# Autodesk Inventor assembly: Assembly_ball_test
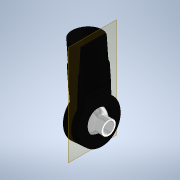
[picture p0: Inventor's stored thumbnail of the model, 180x180]
Saved by Autodesk Inventor 2020 (Build 240168000, 168)
## iProperties
Created: 2019-11-09
Part Number: Assembly_ball_test
Document SubType Name: Assembly
Designer: maste
Author: maste
## Documents named in this file (3)
- C:\Users\maste\Documents\GitHub\autobot\robot_model\Assembly_ball_test.iam
- C:\Users\maste\Documents\GitHub\autobot\robot_model\RCT-H017_Bola_de_libertad_menor.ipt
- C:\Users\maste\Documents\GitHub\autobot\robot_model\RCT-T005_Conexion_superioript.ipt
## Components (2 placed, 2 different names)
1. RCT-H017_Bola_de_libertad_menor:1 — Ball:1
2. RCT-T005_Conexion_superioript:1 — Ball:1, Mate:1
## Relationships (2: BallJoint 1, Mate 1)
- Ball:1: RCT-H017_Bola_de_libertad_menor:1 ↔ RCT-T005_Conexion_superioript:1
- Mate:1: RCT-T005_Conexion_superioript:1
